# Autodesk Inventor assembly: sod_ii_complete
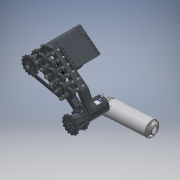
[picture p0: Inventor's stored thumbnail of the model, 180x180]
Saved by Autodesk Inventor 2016 (Build 200138000, 138)
## iProperties
Created: 2016-11-20
Part Number: sod_ii_complete
Document SubType Name: Assembly
Designer: hesaon
Author: hesaon
## Documents named in this file (31)
- D:\documents\SOD-II\cad\sod_ii_complete.iam
- D:\documents\SOD-II\cad\drive_sprocket_middle.ipt
- D:\documents\SOD-II\cad\outer_drive_sprocket.ipt
- D:\documents\SOD-II\cad\screw_Ka22x16.ipt
- D:\documents\SOD-II\cad\motor_axle_mounting_hub_6_mm.ipt
- D:\documents\SOD-II\cad\drive_sprocket_inner.ipt
- D:\documents\SOD-II\cad\screw12x3mm.ipt
- D:\documents\SOD-II\cad\washer3mm.ipt
- D:\documents\SOD-II\cad\tracks_center_ver2.ipt
- D:\documents\SOD-II\cad\tracks_outer.ipt
- D:\documents\SOD-II\cad\37D mm metal gearmotor.ipt
- D:\documents\SOD-II\cad\chassi_front_right.ipt
- D:\documents\SOD-II\cad\chassi_back_right.ipt
- D:\documents\SOD-II\cad\bolt90x6mm.ipt
- D:\documents\SOD-II\cad\washers\washer12mm.ipt
- D:\documents\SOD-II\cad\chassiconnector.ipt
- D:\documents\SOD-II\cad\screws\machine_screw_5_x_24_mm.ipt
- D:\documents\SOD-II\cad\washers\washer_10_mm.ipt
- D:\documents\SOD-II\cad\outer_back_drive_sprocket.ipt
- D:\documents\SOD-II\cad\nuts\nut_5_mm.ipt
- D:\documents\SOD-II\cad\back_sprocket_holder.ipt
- D:\documents\SOD-II\cad\electronics\battery.ipt
- D:\documents\SOD-II\cad\snow_can\snow_can_assembly.iam
- D:\documents\SOD-II\cad\pins\pin_2_x_28_mm.ipt
- D:\documents\SOD-II\cad\tracks\roller_wheel.ipt
- D:\documents\SOD-II\cad\nuts\nut6mm.ipt
- D:\documents\SOD-II\cad\tracks\inner_distance.ipt
- D:\documents\SOD-II\cad\tracks\outer_distance.ipt
- D:\documents\SOD-II\cad\tracks\side_cover.ipt
- D:\documents\SOD-II\cad\back_beam.ipt
- D:\documents\SOD-II\cad\batteryholder.ipt
## Components (185 placed, 29 different names)
1. drive_sprocket_middle:1 — Insert:1, Insert:2, Insert:16, Insert:17
2. outer_drive_sprocket:1 — Insert:1, Insert:2, Insert:3, Insert:4, Insert:5, Insert:6, Insert:7, Insert:8, Insert:9, Insert:10, Insert:11, Insert:12, Insert:13, Insert:14, Insert:43
3. screw_Ka22x16:1 — Insert:6
4. screw_Ka22x16:2 — Insert:4
5. screw_Ka22x16:3 — Insert:3
6. screw_Ka22x16:4 — Insert:7
7. screw_Ka22x16:5 — Insert:10
8. screw_Ka22x16:6 — Insert:9
9. screw_Ka22x16:7 — Insert:8
10. screw_Ka22x16:8 — Insert:5
11. screw_Ka22x16:9 — Insert:14
12. screw_Ka22x16:10 — Insert:11
13. screw_Ka22x16:11 — Insert:12
14. screw_Ka22x16:12 — Insert:13
15. motor_axle_mounting_hub_6_mm:1 — Insert:15, Mate:1, Insert:53
16. drive_sprocket_inner:1 — Insert:15, Mate:1, Insert:16, Insert:17, Insert:25, Insert:26, Insert:27, Insert:28, Insert:29, Insert:30, Insert:31, Insert:32, Insert:33, Insert:34, Insert:35, Insert:36, Insert:37, Insert:38, Insert:39, Insert:40, Insert:41, Insert:42, Insert:44, Insert:45
17. screw12x3mm:1 — Insert:20
18. screw12x3mm:2 — Insert:21
19. screw12x3mm:3 — Insert:22
20. screw12x3mm:4 — Insert:19
21. screw12x3mm:5 — Insert:23
22. screw12x3mm:6 — Insert:24
23. washer3mm:1 — Insert:20, Insert:25
24. washer3mm:2 — Insert:21, Insert:29
25. washer3mm:3 — Insert:22, Insert:28
26. washer3mm:4 — Insert:23, Insert:26
27. washer3mm:5 — Insert:19, Insert:27
28. washer3mm:6 — Insert:24, Insert:30
29. screw_Ka22x16:13 — Insert:40
30. screw_Ka22x16:14 — Insert:33
31. screw_Ka22x16:15 — Insert:34
32. screw_Ka22x16:16 — Insert:31
33. screw_Ka22x16:17 — Insert:39
34. screw_Ka22x16:18 — Insert:37
35. screw_Ka22x16:19 — Insert:42
36. screw_Ka22x16:20 — Insert:32
37. screw_Ka22x16:21 — Insert:36
38. screw_Ka22x16:22 — Insert:38
39. screw_Ka22x16:23 — Insert:41
40. screw_Ka22x16:24 — Insert:35
41. tracks_center_ver2:1 — Insert:45
42. tracks_center_ver2:2 — Insert:44
43. tracks_center_ver2:3 — Insert:43, Insert:48
44. tracks_outer:1 — Insert:48, Insert:50
45. tracks_outer:2 — Insert:49, Insert:50, Insert:51, Insert:52
46. tracks_outer:3 — Insert:49
47. screw_Ka22x16:25 — Insert:52
48. screw_Ka22x16:26 — Insert:51
49. 37D mm metal gearmotor:1 — Insert:53, Insert:54, Insert:55
50. chassi_front_right:1 — Insert:54, Insert:55, Insert:56, Insert:57, Insert:58, Insert:59, Insert:60, Insert:61, Mate:2, Flush:2, Flush:3, Insert:69, Insert:76, Insert:111, Insert:112, Insert:115, Insert:116, Insert:117, Insert:118, Insert:119, Insert:120, Insert:121, Insert:123, Insert:134
51. screw12x3mm:7 — Insert:62
52. screw12x3mm:8 — Insert:64
53. screw12x3mm:9 — Insert:65
54. screw12x3mm:10 — Insert:67
55. screw12x3mm:11 — Insert:66
56. screw12x3mm:12 — Insert:63
57. washer3mm:7 — Insert:56, Insert:63
58. washer3mm:8 — Insert:57, Insert:64
59. washer3mm:9 — Insert:58, Insert:65
60. washer3mm:10 — Insert:61, Insert:67
61. washer3mm:11 — Insert:60, Insert:62
62. washer3mm:12 — Insert:59, Insert:66
63. chassi_back_right:1 — Mate:2, Flush:2, Flush:3, Insert:68, Insert:77, Insert:96, Insert:97, Insert:105, Insert:106, Insert:122, Insert:124, Insert:125, Insert:126, Insert:127, Insert:128, Insert:129, Insert:130, Insert:131, Insert:132, Insert:133, Mate:5, Flush:5, Mate:6, Insert:192, Insert:193
64. bolt90x6mm:1 — Insert:99
65. bolt90x6mm:2 — Insert:98
66. washer12mm:1 — Insert:96, Insert:98
67. washer12mm:2 — Insert:97, Insert:99
68. chassiconnector:1 — Insert:76, Insert:77, Insert:78, Insert:79, Insert:80, Insert:81, Insert:82, Insert:83
69. chassiconnector:2 — Insert:68, Insert:69, Insert:70, Insert:71, Insert:72, Insert:73, Insert:74, Insert:75
70. outer_drive_sprocket:2 — Insert:101, Insert:102, Insert:107
71. outer_drive_sprocket:3 — Insert:101, Insert:102, Insert:103, Insert:104, Insert:108
72. drive_sprocket_middle:2 — Insert:103, Insert:104
73. washer12mm:3 — Insert:109, Insert:110, Insert:191
74. washer12mm:4 — Insert:108, Insert:109
75. washer_10_mm:1 — Insert:70, Insert:89
76. washer_10_mm:2 — Insert:71, Insert:88
77. washer_10_mm:3 — Insert:72, Insert:87
78. washer_10_mm:4 — Insert:73, Insert:84
79. washer_10_mm:5 — Insert:74, Insert:86
80. washer_10_mm:6 — Insert:81, Insert:93
81. washer_10_mm:7 — Insert:83, Insert:95
82. washer_10_mm:8 — Insert:79, Insert:90
83. washer_10_mm:9 — Insert:75, Insert:85
84. washer_10_mm:10 — Insert:78, Insert:91
85. washer_10_mm:11 — Insert:80, Insert:92
86. washer_10_mm:12 — Insert:82, Insert:94
87. machine_screw_5_x_24_mm:1 — Insert:84
88. machine_screw_5_x_24_mm:2 — Insert:85
89. machine_screw_5_x_24_mm:3 — Insert:86
90. machine_screw_5_x_24_mm:4 — Insert:87
91. machine_screw_5_x_24_mm:5 — Insert:88
92. machine_screw_5_x_24_mm:6 — Insert:89
93. nut_5_mm:1 — Insert:94
94. nut_5_mm:2 — Insert:95
95. nut_5_mm:3 — Insert:93
96. nut_5_mm:4 — Insert:90
97. nut_5_mm:5 — Insert:91
98. nut_5_mm:6 — Insert:92
99. bolt90x6mm:3 — Insert:123, Insert:177
100. back_sprocket_holder:1 — Insert:105, Insert:106, Insert:107, Insert:135
101. bolt90x6mm:4 — Insert:122, Insert:176
102. bolt90x6mm:5 — Insert:110
103. battery:1 — Mate:7, Mate:8, Mate:9
104. snow_can_assembly:1 [sub-assembly]
105. washer_10_mm:13 — Insert:111, Insert:113
106. washer_10_mm:14 — Insert:112, Insert:114
107. machine_screw_5_x_24_mm:7 — Insert:113
108. machine_screw_5_x_24_mm:8 — Insert:114
109. pin_2_x_28_mm:1 — Insert:120
110. pin_2_x_28_mm:2 — Insert:119
111. pin_2_x_28_mm:3 — Insert:115
112. pin_2_x_28_mm:4 — Insert:116
113. pin_2_x_28_mm:5 — Insert:117
114. pin_2_x_28_mm:6 — Insert:118
115. pin_2_x_28_mm:7 — Insert:121
116. bolt90x6mm:6 — Insert:125, Insert:174
117. bolt90x6mm:7 — Insert:124, Insert:175
118. bolt90x6mm:8 — Insert:126, Insert:173
119. bolt90x6mm:9 — Insert:127, Insert:172
120. machine_screw_5_x_24_mm:9 — Mate:3
121. washer_10_mm:15 — Insert:128, Mate:3
122. washer12mm:5 — Insert:132, Insert:140
123. washer12mm:6 — Insert:130, Insert:138
124. washer12mm:7 — Insert:131, Insert:139
125. washer12mm:8 — Insert:133, Insert:141
126. washer12mm:9 — Insert:134, Insert:136
127. washer12mm:10 — Insert:135
128. washer12mm:11 — Insert:129, Insert:137
129. nut6mm:1 — Insert:137, Insert:146
130. nut6mm:2 — Insert:136, Insert:147
131. nut6mm:3 — Insert:138, Insert:145
132. nut6mm:4 — Insert:139, Insert:144
133. nut6mm:5 — Insert:140, Insert:143
134. nut6mm:6 — Insert:141, Insert:142
135. inner_distance:1 — Insert:148, Insert:154
136. inner_distance:2 — Insert:149, Insert:155
137. inner_distance:3 — Insert:150, Insert:156
138. inner_distance:4 — Insert:151, Insert:157
139. inner_distance:5 — Insert:152, Insert:158
140. inner_distance:6 — Insert:153, Insert:159
141. washer12mm:12 — Insert:147, Insert:153
142. washer12mm:13 — Insert:146, Insert:152
143. washer12mm:14 — Insert:145, Insert:151
144. washer12mm:15 — Insert:144, Insert:150
145. washer12mm:16 — Insert:142, Insert:148
146. washer12mm:17 — Insert:143, Insert:149
147. washer12mm:18 — Insert:159, Insert:163
148. washer12mm:19 — Insert:158, Insert:162
149. washer12mm:20 — Insert:157, Insert:164
150. washer12mm:21 — Insert:156, Insert:161
151. washer12mm:22 — Insert:155, Insert:165
152. washer12mm:23 — Insert:154, Insert:160
153. roller_wheel:5 — Insert:163, Insert:166
154. roller_wheel:6 — Insert:165, Insert:170
155. roller_wheel:7 — Insert:162, Insert:167
156. roller_wheel:8 — Insert:161, Insert:169
157. roller_wheel:9 — Insert:164, Insert:168
158. roller_wheel:10 — Insert:160, Insert:171
159. washer12mm:24 — Insert:170, Insert:185
160. washer12mm:25 — Insert:168, Insert:187
161. washer12mm:26 — Insert:167, Insert:188
162. washer12mm:27 — Insert:166, Insert:189
163. washer12mm:28 — Insert:171, Insert:184
164. washer12mm:29 — Insert:169, Insert:186
165. washer12mm:30 — Insert:172, Insert:178
166. washer12mm:31 — Insert:173, Insert:179
167. washer12mm:32 — Insert:174, Insert:180
168. washer12mm:33 — Insert:175, Insert:181
169. washer12mm:34 — Insert:176, Insert:182
170. washer12mm:35 — Insert:177, Insert:183, Insert:190
171. washer12mm:36 — Insert:183
172. washer12mm:37 — Insert:182
173. washer12mm:38 — Insert:181
174. washer12mm:39 — Insert:180
175. washer12mm:40 — Insert:179
176. washer12mm:41 — Insert:178
177. outer_distance:1 — Insert:185
178. outer_distance:2 — Insert:186
179. outer_distance:3 — Insert:184
180. outer_distance:4 — Insert:187
181. outer_distance:5 — Insert:188
182. outer_distance:6 — Insert:189
183. side_cover:1 — Insert:190, Insert:191
184. back_beam:1 — Mate:5, Flush:5, Mate:6
185. batteryholder:1 — Insert:192, Insert:193, Mate:7, Mate:8, Mate:9
## Relationships (200: Insert 189, Mate 8, Flush 3)
- Insert:1: drive_sprocket_middle:1 ↔ outer_drive_sprocket:1
- Insert:2: drive_sprocket_middle:1 ↔ outer_drive_sprocket:1
- Insert:3: outer_drive_sprocket:1 ↔ screw_Ka22x16:3
- Insert:4: outer_drive_sprocket:1 ↔ screw_Ka22x16:2
- Insert:5: outer_drive_sprocket:1 ↔ screw_Ka22x16:8
- Insert:6: outer_drive_sprocket:1 ↔ screw_Ka22x16:1
- Insert:7: outer_drive_sprocket:1 ↔ screw_Ka22x16:4
- Insert:8: outer_drive_sprocket:1 ↔ screw_Ka22x16:7
- Insert:9: outer_drive_sprocket:1 ↔ screw_Ka22x16:6
- Insert:10: outer_drive_sprocket:1 ↔ screw_Ka22x16:5
- Insert:11: outer_drive_sprocket:1 ↔ screw_Ka22x16:10
- Insert:12: outer_drive_sprocket:1 ↔ screw_Ka22x16:11
- Insert:13: outer_drive_sprocket:1 ↔ screw_Ka22x16:12
- Insert:14: outer_drive_sprocket:1 ↔ screw_Ka22x16:9
- Insert:15: motor_axle_mounting_hub_6_mm:1 ↔ drive_sprocket_inner:1
- Mate:1: motor_axle_mounting_hub_6_mm:1 ↔ drive_sprocket_inner:1
- Insert:16: drive_sprocket_middle:1 ↔ drive_sprocket_inner:1
- Insert:17: drive_sprocket_middle:1 ↔ drive_sprocket_inner:1
- Insert:19: screw12x3mm:4 ↔ washer3mm:5
- Insert:20: screw12x3mm:1 ↔ washer3mm:1
- Insert:21: screw12x3mm:2 ↔ washer3mm:2
- Insert:22: screw12x3mm:3 ↔ washer3mm:3
- Insert:23: screw12x3mm:5 ↔ washer3mm:4
- Insert:24: screw12x3mm:6 ↔ washer3mm:6
- Insert:25: drive_sprocket_inner:1 ↔ washer3mm:1
- Insert:26: drive_sprocket_inner:1 ↔ washer3mm:4
- Insert:27: drive_sprocket_inner:1 ↔ washer3mm:5
- Insert:28: drive_sprocket_inner:1 ↔ washer3mm:3
- Insert:29: drive_sprocket_inner:1 ↔ washer3mm:2
- Insert:30: drive_sprocket_inner:1 ↔ washer3mm:6
- Insert:31: drive_sprocket_inner:1 ↔ screw_Ka22x16:16
- Insert:32: drive_sprocket_inner:1 ↔ screw_Ka22x16:20
- Insert:33: drive_sprocket_inner:1 ↔ screw_Ka22x16:14
- Insert:34: drive_sprocket_inner:1 ↔ screw_Ka22x16:15
- Insert:35: drive_sprocket_inner:1 ↔ screw_Ka22x16:24
- Insert:36: drive_sprocket_inner:1 ↔ screw_Ka22x16:21
- Insert:37: drive_sprocket_inner:1 ↔ screw_Ka22x16:18
- Insert:38: drive_sprocket_inner:1 ↔ screw_Ka22x16:22
- Insert:39: drive_sprocket_inner:1 ↔ screw_Ka22x16:17
- Insert:40: drive_sprocket_inner:1 ↔ screw_Ka22x16:13
- Insert:41: drive_sprocket_inner:1 ↔ screw_Ka22x16:23
- Insert:42: drive_sprocket_inner:1 ↔ screw_Ka22x16:19
- Insert:43 (-0.2925 mm): outer_drive_sprocket:1 ↔ tracks_center_ver2:3
- Insert:44 (-0.2925 mm): drive_sprocket_inner:1 ↔ tracks_center_ver2:2
- Insert:45 (-0.2925 mm): drive_sprocket_inner:1 ↔ tracks_center_ver2:1
- Insert:48: tracks_center_ver2:3 ↔ tracks_outer:1
- Insert:49: tracks_outer:2 ↔ tracks_outer:3
- Insert:50: tracks_outer:1 ↔ tracks_outer:2
- Insert:51: tracks_outer:2 ↔ screw_Ka22x16:26
- Insert:52: tracks_outer:2 ↔ screw_Ka22x16:25
- Insert:53: motor_axle_mounting_hub_6_mm:1 ↔ 37D mm metal gearmotor:1
- Insert:54: 37D mm metal gearmotor:1 ↔ chassi_front_right:1
- Insert:55: 37D mm metal gearmotor:1 ↔ chassi_front_right:1
- Insert:56: chassi_front_right:1 ↔ washer3mm:7
- Insert:57: chassi_front_right:1 ↔ washer3mm:8
- Insert:58: chassi_front_right:1 ↔ washer3mm:9
- Insert:59: chassi_front_right:1 ↔ washer3mm:12
- Insert:60: chassi_front_right:1 ↔ washer3mm:11
- Insert:61: chassi_front_right:1 ↔ washer3mm:10
- Insert:62: screw12x3mm:7 ↔ washer3mm:11
- Insert:63: screw12x3mm:12 ↔ washer3mm:7
- Insert:64: screw12x3mm:8 ↔ washer3mm:8
- Insert:65: screw12x3mm:9 ↔ washer3mm:9
- Insert:66: screw12x3mm:11 ↔ washer3mm:12
- Insert:67: screw12x3mm:10 ↔ washer3mm:10
- Mate:2: chassi_front_right:1 ↔ chassi_back_right:1
- Flush:2: chassi_front_right:1 ↔ chassi_back_right:1
- Flush:3: chassi_front_right:1 ↔ chassi_back_right:1
- Insert:68: chassi_back_right:1 ↔ chassiconnector:2
- Insert:69: chassi_front_right:1 ↔ chassiconnector:2
- Insert:70: chassiconnector:2 ↔ washer_10_mm:1
- Insert:71: chassiconnector:2 ↔ washer_10_mm:2
- Insert:72: chassiconnector:2 ↔ washer_10_mm:3
- Insert:73: chassiconnector:2 ↔ washer_10_mm:4
- Insert:74: chassiconnector:2 ↔ washer_10_mm:5
- Insert:75: chassiconnector:2 ↔ washer_10_mm:9
- Insert:76: chassi_front_right:1 ↔ chassiconnector:1
- Insert:77: chassi_back_right:1 ↔ chassiconnector:1
- Insert:78: chassiconnector:1 ↔ washer_10_mm:10
- Insert:79: chassiconnector:1 ↔ washer_10_mm:8
- Insert:80: chassiconnector:1 ↔ washer_10_mm:11
- Insert:81: chassiconnector:1 ↔ washer_10_mm:6
- Insert:82: chassiconnector:1 ↔ washer_10_mm:12
- Insert:83: chassiconnector:1 ↔ washer_10_mm:7
- Insert:84: washer_10_mm:4 ↔ machine_screw_5_x_24_mm:1
- Insert:85: washer_10_mm:9 ↔ machine_screw_5_x_24_mm:2
- Insert:86: washer_10_mm:5 ↔ machine_screw_5_x_24_mm:3
- Insert:87: washer_10_mm:3 ↔ machine_screw_5_x_24_mm:4
- Insert:88: washer_10_mm:2 ↔ machine_screw_5_x_24_mm:5
- Insert:89: washer_10_mm:1 ↔ machine_screw_5_x_24_mm:6
- Insert:90: washer_10_mm:8 ↔ nut_5_mm:4
- Insert:91: washer_10_mm:10 ↔ nut_5_mm:5
- Insert:92: washer_10_mm:11 ↔ nut_5_mm:6
- Insert:93: washer_10_mm:6 ↔ nut_5_mm:3
- Insert:94: washer_10_mm:12 ↔ nut_5_mm:1
- Insert:95: washer_10_mm:7 ↔ nut_5_mm:2
- Insert:96: chassi_back_right:1 ↔ washer12mm:1
- Insert:97: chassi_back_right:1 ↔ washer12mm:2
- Insert:98: bolt90x6mm:2 ↔ washer12mm:1
- Insert:99: bolt90x6mm:1 ↔ washer12mm:2
- Insert:101 (30 mm): outer_drive_sprocket:2 ↔ outer_drive_sprocket:3
- Insert:102 (30 mm): outer_drive_sprocket:2 ↔ outer_drive_sprocket:3
- Insert:103: outer_drive_sprocket:3 ↔ drive_sprocket_middle:2
- Insert:104: outer_drive_sprocket:3 ↔ drive_sprocket_middle:2
- Insert:105: chassi_back_right:1 ↔ back_sprocket_holder:1
- Insert:106: chassi_back_right:1 ↔ back_sprocket_holder:1
- Insert:107 (21 mm): outer_drive_sprocket:2 ↔ back_sprocket_holder:1
- Insert:108: outer_drive_sprocket:3 ↔ washer12mm:4
- Insert:109 (3 mm): washer12mm:3 ↔ washer12mm:4
- Insert:110: washer12mm:3 ↔ bolt90x6mm:5
- Insert:111: chassi_front_right:1 ↔ washer_10_mm:13
- Insert:112: chassi_front_right:1 ↔ washer_10_mm:14
- Insert:113: washer_10_mm:13 ↔ machine_screw_5_x_24_mm:7
- Insert:114: washer_10_mm:14 ↔ machine_screw_5_x_24_mm:8
- Insert:115: chassi_front_right:1 ↔ pin_2_x_28_mm:3
- Insert:116: chassi_front_right:1 ↔ pin_2_x_28_mm:4
- Insert:117: chassi_front_right:1 ↔ pin_2_x_28_mm:5
- Insert:118: chassi_front_right:1 ↔ pin_2_x_28_mm:6
- Insert:119: chassi_front_right:1 ↔ pin_2_x_28_mm:2
- Insert:120: chassi_front_right:1 ↔ pin_2_x_28_mm:1
- Insert:121: chassi_front_right:1 ↔ pin_2_x_28_mm:7
- Insert:122 (-17.185 mm): chassi_back_right:1 ↔ bolt90x6mm:4
- Insert:123 (-17.185 mm): chassi_front_right:1 ↔ bolt90x6mm:3
- Insert:124 (-17.185 mm): chassi_back_right:1 ↔ bolt90x6mm:7
- Insert:125 (-17.185 mm): chassi_back_right:1 ↔ bolt90x6mm:6
- Insert:126 (-17.185 mm): chassi_back_right:1 ↔ bolt90x6mm:8
- Insert:127 (-17.185 mm): chassi_back_right:1 ↔ bolt90x6mm:9
- Insert:128: chassi_back_right:1 ↔ washer_10_mm:15
- Mate:3: machine_screw_5_x_24_mm:9 ↔ washer_10_mm:15
- Insert:129: chassi_back_right:1 ↔ washer12mm:11
- Insert:130: chassi_back_right:1 ↔ washer12mm:6
- Insert:131: chassi_back_right:1 ↔ washer12mm:7
- Insert:132: chassi_back_right:1 ↔ washer12mm:5
- Insert:133: chassi_back_right:1 ↔ washer12mm:8
- Insert:134: chassi_front_right:1 ↔ washer12mm:9
- Insert:135: back_sprocket_holder:1 ↔ washer12mm:10
- Insert:136: washer12mm:9 ↔ nut6mm:2
- Insert:137: washer12mm:11 ↔ nut6mm:1
- Insert:138: washer12mm:6 ↔ nut6mm:3
- Insert:139: washer12mm:7 ↔ nut6mm:4
- Insert:140: washer12mm:5 ↔ nut6mm:5
- Insert:141: washer12mm:8 ↔ nut6mm:6
- Insert:142: nut6mm:6 ↔ washer12mm:16
- Insert:143: nut6mm:5 ↔ washer12mm:17
- Insert:144: nut6mm:4 ↔ washer12mm:15
- Insert:145: nut6mm:3 ↔ washer12mm:14
- Insert:146: nut6mm:1 ↔ washer12mm:13
- Insert:147: nut6mm:2 ↔ washer12mm:12
- Insert:148: inner_distance:1 ↔ washer12mm:16
- Insert:149: inner_distance:2 ↔ washer12mm:17
- Insert:150: inner_distance:3 ↔ washer12mm:15
- Insert:151: inner_distance:4 ↔ washer12mm:14
- Insert:152: inner_distance:5 ↔ washer12mm:13
- Insert:153: inner_distance:6 ↔ washer12mm:12
- Insert:154: inner_distance:1 ↔ washer12mm:23
- Insert:155: inner_distance:2 ↔ washer12mm:22
- Insert:156: inner_distance:3 ↔ washer12mm:21
- Insert:157: inner_distance:4 ↔ washer12mm:20
- Insert:158: inner_distance:5 ↔ washer12mm:19
- Insert:159: inner_distance:6 ↔ washer12mm:18
- Insert:160: washer12mm:23 ↔ roller_wheel:10
- Insert:161: washer12mm:21 ↔ roller_wheel:8
- Insert:162: washer12mm:19 ↔ roller_wheel:7
- Insert:163: washer12mm:18 ↔ roller_wheel:5
- Insert:164: washer12mm:20 ↔ roller_wheel:9
- Insert:165: washer12mm:22 ↔ roller_wheel:6
- Insert:166: roller_wheel:5 ↔ washer12mm:27
- Insert:167: roller_wheel:7 ↔ washer12mm:26
- Insert:168: roller_wheel:9 ↔ washer12mm:25
- Insert:169: roller_wheel:8 ↔ washer12mm:29
- Insert:170: roller_wheel:6 ↔ washer12mm:24
- Insert:171: roller_wheel:10 ↔ washer12mm:28
- Insert:172: bolt90x6mm:9 ↔ washer12mm:30
- Insert:173: bolt90x6mm:8 ↔ washer12mm:31
- Insert:174: bolt90x6mm:6 ↔ washer12mm:32
- Insert:175: bolt90x6mm:7 ↔ washer12mm:33
- Insert:176: bolt90x6mm:4 ↔ washer12mm:34
- Insert:177: bolt90x6mm:3 ↔ washer12mm:35
- Insert:178 (3 mm): washer12mm:30 ↔ washer12mm:41
- Insert:179 (3 mm): washer12mm:31 ↔ washer12mm:40
- Insert:180 (3 mm): washer12mm:32 ↔ washer12mm:39
- Insert:181 (3 mm): washer12mm:33 ↔ washer12mm:38
- Insert:182 (3 mm): washer12mm:34 ↔ washer12mm:37
- Insert:183 (3 mm): washer12mm:35 ↔ washer12mm:36
- Insert:184: washer12mm:28 ↔ outer_distance:3
- Insert:185: washer12mm:24 ↔ outer_distance:1
- Insert:186: washer12mm:29 ↔ outer_distance:2
- Insert:187: washer12mm:25 ↔ outer_distance:4
- Insert:188: washer12mm:26 ↔ outer_distance:5
- Insert:189: washer12mm:27 ↔ outer_distance:6
- Insert:190: washer12mm:35 ↔ side_cover:1
- Insert:191: washer12mm:3 ↔ side_cover:1
- Mate:5: chassi_back_right:1 ↔ back_beam:1
- Flush:5: chassi_back_right:1 ↔ back_beam:1
- Mate:6: chassi_back_right:1 ↔ back_beam:1
- Insert:192: chassi_back_right:1 ↔ batteryholder:1
- Insert:193: chassi_back_right:1 ↔ batteryholder:1
- Mate:7: battery:1 ↔ batteryholder:1
- Mate:8: battery:1 ↔ batteryholder:1
- Mate:9: battery:1 ↔ batteryholder:1
